# Autodesk Inventor assembly: wall_shelf
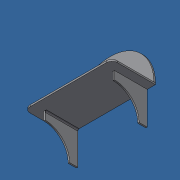
[picture p0: Inventor's stored thumbnail of the model, 180x180]
Saved by Autodesk Inventor 2022.4 (Build 264492010, 492A)
## iProperties
Created: 2007-01-12
Part Number: wall_shelf
Document SubType Name: Weldment
Designer: ceirmann
Weld Material: Welded Aluminum-6061
Mass: 1298.65 g
Surface Area: 3805.3 cm^2
Volume: 1289.86 cm^3
Density: 1.00682 g/cm^3
CN_MASS: 1.3
Author: ceirmann
## Documents named in this file (4)
- U:\Inventor 2022 Training\_Designer Training\Inventor 2022 - Advanced Assembly\Practice Files\wall_shelf.iam
- U:\Inventor 2022 Training\_Designer Training\Inventor 2022 - Advanced Assembly\Practice Files\support.ipt
- U:\Inventor 2022 Training\_Designer Training\Inventor 2022 - Advanced Assembly\Practice Files\slab.ipt
- U:\Inventor 2022 Training\_Designer Training\Inventor 2022 - Advanced Assembly\Practice Files\shelf-backplate.ipt
## Components (4 placed, 3 different names)
1. slab:1 — Flush:1, Mate:1, Flush:2, Flush:3, Mate:2, Flush:4, Mate:3, Flush:5, Mate:4
2. support:1 — Flush:1, Mate:1, Flush:2
3. support:2 — Flush:3, Mate:2, Flush:4
4. shelf-backplate:1 — Mate:3, Flush:5, Mate:4
## Relationships (9: Flush 5, Mate 4)
- Flush:1: slab:1 ↔ support:1
- Mate:1: slab:1 ↔ support:1
- Flush:2 (-38.1 mm): slab:1 ↔ support:1
- Flush:3: slab:1 ↔ support:2
- Mate:2: slab:1 ↔ support:2
- Flush:4 (-38.1 mm): slab:1 ↔ support:2
- Mate:3: slab:1 ↔ shelf-backplate:1
- Flush:5: slab:1 ↔ shelf-backplate:1
- Mate:4: slab:1 ↔ shelf-backplate:1
